# Autodesk Inventor assembly: Assembly3
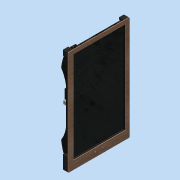
[picture p0: Inventor's stored thumbnail of the model, 180x180]
Saved by Autodesk Inventor 2017 (Build 210142000, 142)
## iProperties
Created: 2018-10-04
Part Number: Assembly3
Document SubType Name: Assembly
Designer: mailb
Author: mailb
## Documents named in this file (12)
- C:\Users\mailb\Documents\Inventor\MirageSmartMirror\Assembly3.iam
- C:\Users\mailb\Documents\Inventor\MirageSmartMirror\DellP2317H.ipt
- C:\Users\mailb\Documents\Inventor\MirageSmartMirror\RPi3B.ipt
- C:\Users\mailb\Documents\Inventor\MirageSmartMirror\RPiCamV2.iam
- C:\Users\mailb\Documents\Inventor\MirageSmartMirror\Part23.ipt
- C:\Users\mailb\Documents\Inventor\MirageSmartMirror\APDS9960.iam
- C:\Users\mailb\Documents\Inventor\MirageSmartMirror\Part68.ipt
- C:\Users\mailb\Documents\Inventor\MirageSmartMirror\Part69.ipt
- C:\Users\mailb\Documents\Inventor\MirageSmartMirror\Part69_MIR.ipt
- C:\Users\mailb\Documents\Inventor\MirageSmartMirror\Part1.ipt
- C:\Users\mailb\Documents\Inventor\MirageSmartMirror\Part1_MIR.ipt
- C:\Users\mailb\Documents\Inventor\MirageSmartMirror\Part3.ipt
## Components (11 placed, 11 different names)
1. DellP2317H:1 — Mate:1, Flush:1, Flush:2, Mate:2, Flush:3, Flush:4, Flush:5, Mate:3, Flush:7, Mate:5, Mate:6, Mate:8, Mate:9
2. RPi3B:1 — Mate:1, Flush:1, Flush:2
3. RPiCamV2:1 [sub-assembly] — Mate:2, Flush:3, Flush:4, Flush:9
4. Part23:1 — Flush:5, Flush:8, Flush:9, Flush:10, Flush:11, Flush:12, Flush:13, Mate:4, Flush:14, Flush:15, Mate:7, Flush:16, Flush:17
5. APDS9960:1 [sub-assembly] — Mate:3, Flush:7, Flush:8
6. Part68:1 — Flush:10, Flush:11
7. Part69:1 — Flush:12, Flush:13
8. Part69_MIR:1 — Mate:4, Mate:5, Mate:6
9. Part1:1 — Flush:14, Flush:15
10. Part1_MIR:1 — Mate:7, Mate:8, Mate:9
11. Part3:1 — Flush:16, Flush:17
## Relationships (25: Flush 16, Mate 9)
- Mate:1: DellP2317H:1 ↔ RPi3B:1
- Flush:1: DellP2317H:1 ↔ RPi3B:1
- Flush:2 (177.8 mm): DellP2317H:1 ↔ RPi3B:1
- Mate:2: DellP2317H:1 ↔ RPiCamV2:1
- Flush:3: DellP2317H:1 ↔ RPiCamV2:1
- Flush:4 (127 mm): DellP2317H:1 ↔ RPiCamV2:1
- Flush:5: DellP2317H:1 ↔ Part23:1
- Mate:3: DellP2317H:1 ↔ APDS9960:1
- Flush:7 (127 mm): DellP2317H:1 ↔ APDS9960:1
- Flush:8: Part23:1 ↔ APDS9960:1
- Flush:9: RPiCamV2:1 ↔ Part23:1
- Flush:10: Part23:1 ↔ Part68:1
- Flush:11: Part23:1 ↔ Part68:1
- Flush:12: Part23:1 ↔ Part69:1
- Flush:13: Part23:1 ↔ Part69:1
- Mate:4: Part23:1 ↔ Part69_MIR:1
- Mate:5: DellP2317H:1 ↔ Part69_MIR:1
- Mate:6: DellP2317H:1 ↔ Part69_MIR:1
- Flush:14: Part23:1 ↔ Part1:1
- Flush:15: Part23:1 ↔ Part1:1
- Mate:7: Part23:1 ↔ Part1_MIR:1
- Mate:8: DellP2317H:1 ↔ Part1_MIR:1
- Mate:9: DellP2317H:1 ↔ Part1_MIR:1
- Flush:16: Part23:1 ↔ Part3:1
- Flush:17: Part23:1 ↔ Part3:1
